# Autodesk Inventor assembly: Robot4
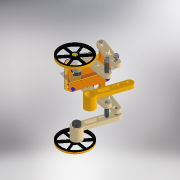
[picture p0: Inventor's stored thumbnail of the model, 180x180]
Saved by Autodesk Inventor 2021 (Build 250183000, 183)
## iProperties
Created: 2024-04-10
Part Number: Robot4
Document SubType Name: Assembly
Designer: Martin
Author: Martin
## Documents named in this file (17)
- C:\Users\ASUS\OneDrive - Universidad de Antioquia\2024-1\Robótica\Proyecto\CAD\op1\Robot4.iam
- C:\Users\ASUS\OneDrive - Universidad de Antioquia\2024-1\Robótica\Proyecto\CAD\op1\BaseEnsamble.iam
- C:\Users\ASUS\OneDrive - Universidad de Antioquia\2024-1\Robótica\Proyecto\CAD\op1\EslabonCodoTrasero.ipt
- C:\Users\ASUS\OneDrive - Universidad de Antioquia\2024-1\Robótica\Proyecto\CAD\op1\EslabonRodillaCadera.ipt
- C:\Users\ASUS\OneDrive - Universidad de Antioquia\2024-1\Robótica\Proyecto\CAD\op1\Llana.ipt
- C:\Users\ASUS\OneDrive - Universidad de Antioquia\2024-1\Robótica\Proyecto\CAD\37d-gearmotor-19-30-encoder.ipt
- C:\Users\ASUS\OneDrive - Universidad de Antioquia\2024-1\Robótica\Proyecto\CAD\Resorte.ipt
- C:\Users\ASUS\Documents\Inventor\Content Center Files\R2021\en-US\GB_T 276-94 60000-RS and LS\Bearing 61900-LS GB_T 276-94.ipt
- C:\Users\ASUS\Documents\Inventor\Content Center Files\R2021\en-US\AS 1111\AS 1111 - M8 x 90.ipt
- C:\Users\ASUS\Documents\Inventor\Content Center Files\R2021\en-US\ISO 1207(2)\ISO 1207 - M8 x 50.ipt
- C:\Users\ASUS\Documents\Inventor\Content Center Files\R2021\en-US\AS 1112 (2)\AS 1112 - M8  Type 5.ipt
- C:\Users\ASUS\OneDrive - Universidad de Antioquia\2024-1\Robótica\Proyecto\CAD\op1\EslabonCodoTrasero_MIR2.ipt
- C:\Users\ASUS\OneDrive - Universidad de Antioquia\2024-1\Robótica\Proyecto\CAD\op1\EslabonRodillaCadera_MIR2.ipt
- C:\Users\ASUS\OneDrive - Universidad de Antioquia\2024-1\Robótica\Proyecto\CAD\op1\EslabonRuedaRodilla_MIR2.ipt
- C:\Users\ASUS\OneDrive - Universidad de Antioquia\2024-1\Robótica\Proyecto\CAD\op1\Llana_MIR1.ipt
- C:\Users\ASUS\OneDrive - Universidad de Antioquia\2024-1\Robótica\Proyecto\CAD\37d-gearmotor-19-30-encoder_MIR2.ipt
- C:\Users\ASUS\OneDrive - Universidad de Antioquia\2024-1\Robótica\Proyecto\CAD\Resorte_MIR3.ipt
## Components (39 placed, 16 different names)
1. BaseEnsamble:1 [sub-assembly] — Mate:11, Mate:12, Mate:13, Insert:1
2. EslabonCodoTrasero:1 — Mate:13, Mate:22, Mate:23, Mate:28, Mate:29, Insert:2, Insert:3
3. EslabonRodillaCadera:1 — Mate:11, Mate:12, Mate:14, Mate:15
4. Llana:1 — Mate:5
5. 37d-gearmotor-19-30-encoder:1 — Mate:5
6. Resorte:1
7. Rolling bearing GB/T 276-1994 Type 60000-RS and LS 61900-LS:1 — Mate:14, Mate:15
8. Rolling bearing GB/T 276-1994 Type 60000-RS and LS 61900-LS:2
9. Rolling bearing GB/T 276-1994 Type 60000-RS and LS 61900-LS:3 — Mate:22, Mate:23, Mate:31
10. Rolling bearing GB/T 276-1994 Type 60000-RS and LS 61900-LS:4
11. Rolling bearing GB/T 276-1994 Type 60000-RS and LS 61900-LS:5
12. AS 1111 - Metric M8 x 90:1 — Mate:32
13. ISO 1207 M8 x 50:1 — Mate:30
14. AS 1111 - Metric M8 x 90:2 — Mate:28, Mate:29
15. AS 1112 (2) - Metric M8  Type 5:1 — Insert:1
16. AS 1112 (2) - Metric M8  Type 5:2 — Mate:30, Mate:31
17. AS 1112 (2) - Metric M8  Type 5:3 — Insert:2
18. AS 1112 (2) - Metric M8  Type 5:4 — Insert:3
19. AS 1112 (2) - Metric M8  Type 5:5 — Mate:32
20. EslabonCodoTrasero_MIR2:1 — Mate:33, Mate:34, Mate:46, Mate:47, Mate:56, Mate:57, Insert:4, Insert:5
21. EslabonRodillaCadera_MIR2:1 — Mate:35, Mate:36, Mate:42, Mate:43
22. EslabonRuedaRodilla_MIR2:1 — Mate:33, Mate:34, Mate:35, Mate:36, Mate:37, Mate:39, Mate:40, Mate:41, Mate:44, Mate:45, Mate:48, Mate:49, Mate:50, Mate:51, Mate:52, Mate:53, Mate:54, Mate:55
23. Llana_MIR1:1 — Mate:37, Mate:38
24. 37d-gearmotor-19-30-encoder_MIR2:1 — Mate:38, Mate:39, Mate:40
25. Resorte_MIR3:1 — Mate:41
26. Rolling bearing GB/T 276-1994 Type 60000-RS and LS 61900-LS:6 — Mate:42, Mate:43
27. Rolling bearing GB/T 276-1994 Type 60000-RS and LS 61900-LS:7 — Mate:44, Mate:45
28. Rolling bearing GB/T 276-1994 Type 60000-RS and LS 61900-LS:8 — Mate:46, Mate:47, Mate:58
29. Rolling bearing GB/T 276-1994 Type 60000-RS and LS 61900-LS:9 — Mate:48, Mate:49
30. Rolling bearing GB/T 276-1994 Type 60000-RS and LS 61900-LS:10 — Mate:50, Mate:51
31. AS 1111 - Metric M8 x 90:3 — Mate:52, Mate:53, Mate:60
32. ISO 1207 M8 x 50:2 — Mate:54, Mate:55, Mate:59
33. AS 1111 - Metric M8 x 90:4 — Mate:56, Mate:57
34. AS 1112 (2) - Metric M8  Type 5:6
35. AS 1112 (2) - Metric M8  Type 5:7 — Mate:58, Mate:59
36. AS 1112 (2) - Metric M8  Type 5:8 — Insert:4
37. AS 1112 (2) - Metric M8  Type 5:9 — Insert:5
38. AS 1112 (2) - Metric M8  Type 5:10 — Mate:60
39. EslabonRuedaRodilla_MIR2:2
## Relationships (46: Mate 41, Insert 5)
- Mate:5: Llana:1 ↔ 37d-gearmotor-19-30-encoder:1
- Mate:11: BaseEnsamble:1 ↔ EslabonRodillaCadera:1
- Mate:12 (1 mm): BaseEnsamble:1 ↔ EslabonRodillaCadera:1
- Mate:13: BaseEnsamble:1 ↔ EslabonCodoTrasero:1
- Mate:14: EslabonRodillaCadera:1 ↔ Rolling bearing GB/T 276-1994 Type 60000-RS and LS 61900-LS:1
- Mate:15: EslabonRodillaCadera:1 ↔ Rolling bearing GB/T 276-1994 Type 60000-RS and LS 61900-LS:1
- Mate:22: EslabonCodoTrasero:1 ↔ Rolling bearing GB/T 276-1994 Type 60000-RS and LS 61900-LS:3
- Mate:23: EslabonCodoTrasero:1 ↔ Rolling bearing GB/T 276-1994 Type 60000-RS and LS 61900-LS:3
- Mate:28: EslabonCodoTrasero:1 ↔ AS 1111 - Metric M8 x 90:2
- Mate:29: EslabonCodoTrasero:1 ↔ AS 1111 - Metric M8 x 90:2
- Insert:1: BaseEnsamble:1 ↔ AS 1112 (2) - Metric M8  Type 5:1
- Mate:30: ISO 1207 M8 x 50:1 ↔ AS 1112 (2) - Metric M8  Type 5:2
- Mate:31: Rolling bearing GB/T 276-1994 Type 60000-RS and LS 61900-LS:3 ↔ AS 1112 (2) - Metric M8  Type 5:2
- Insert:2: EslabonCodoTrasero:1 ↔ AS 1112 (2) - Metric M8  Type 5:3
- Insert:3: EslabonCodoTrasero:1 ↔ AS 1112 (2) - Metric M8  Type 5:4
- Mate:32: AS 1111 - Metric M8 x 90:1 ↔ AS 1112 (2) - Metric M8  Type 5:5
- Mate:33 (10 mm): EslabonCodoTrasero_MIR2:1 ↔ EslabonRuedaRodilla_MIR2:1
- Mate:34: EslabonCodoTrasero_MIR2:1 ↔ EslabonRuedaRodilla_MIR2:1
- Mate:35 (46 mm): EslabonRodillaCadera_MIR2:1 ↔ EslabonRuedaRodilla_MIR2:1
- Mate:36: EslabonRodillaCadera_MIR2:1 ↔ EslabonRuedaRodilla_MIR2:1
- Mate:37 (2 mm): EslabonRuedaRodilla_MIR2:1 ↔ Llana_MIR1:1
- Mate:38: Llana_MIR1:1 ↔ 37d-gearmotor-19-30-encoder_MIR2:1
- Mate:39: EslabonRuedaRodilla_MIR2:1 ↔ 37d-gearmotor-19-30-encoder_MIR2:1
- Mate:40: EslabonRuedaRodilla_MIR2:1 ↔ 37d-gearmotor-19-30-encoder_MIR2:1
- Mate:41: EslabonRuedaRodilla_MIR2:1 ↔ Resorte_MIR3:1
- Mate:42: EslabonRodillaCadera_MIR2:1 ↔ Rolling bearing GB/T 276-1994 Type 60000-RS and LS 61900-LS:6
- Mate:43: EslabonRodillaCadera_MIR2:1 ↔ Rolling bearing GB/T 276-1994 Type 60000-RS and LS 61900-LS:6
- Mate:44: EslabonRuedaRodilla_MIR2:1 ↔ Rolling bearing GB/T 276-1994 Type 60000-RS and LS 61900-LS:7
- Mate:45: EslabonRuedaRodilla_MIR2:1 ↔ Rolling bearing GB/T 276-1994 Type 60000-RS and LS 61900-LS:7
- Mate:46: EslabonCodoTrasero_MIR2:1 ↔ Rolling bearing GB/T 276-1994 Type 60000-RS and LS 61900-LS:8
- Mate:47: EslabonCodoTrasero_MIR2:1 ↔ Rolling bearing GB/T 276-1994 Type 60000-RS and LS 61900-LS:8
- Mate:48: EslabonRuedaRodilla_MIR2:1 ↔ Rolling bearing GB/T 276-1994 Type 60000-RS and LS 61900-LS:9
- Mate:49: EslabonRuedaRodilla_MIR2:1 ↔ Rolling bearing GB/T 276-1994 Type 60000-RS and LS 61900-LS:9
- Mate:50: EslabonRuedaRodilla_MIR2:1 ↔ Rolling bearing GB/T 276-1994 Type 60000-RS and LS 61900-LS:10
- Mate:51: EslabonRuedaRodilla_MIR2:1 ↔ Rolling bearing GB/T 276-1994 Type 60000-RS and LS 61900-LS:10
- Mate:52: EslabonRuedaRodilla_MIR2:1 ↔ AS 1111 - Metric M8 x 90:3
- Mate:53: EslabonRuedaRodilla_MIR2:1 ↔ AS 1111 - Metric M8 x 90:3
- Mate:54: EslabonRuedaRodilla_MIR2:1 ↔ ISO 1207 M8 x 50:2
- Mate:55: EslabonRuedaRodilla_MIR2:1 ↔ ISO 1207 M8 x 50:2
- Mate:56: EslabonCodoTrasero_MIR2:1 ↔ AS 1111 - Metric M8 x 90:4
- Mate:57: EslabonCodoTrasero_MIR2:1 ↔ AS 1111 - Metric M8 x 90:4
- Mate:58: Rolling bearing GB/T 276-1994 Type 60000-RS and LS 61900-LS:8 ↔ AS 1112 (2) - Metric M8  Type 5:7
- Mate:59: ISO 1207 M8 x 50:2 ↔ AS 1112 (2) - Metric M8  Type 5:7
- Insert:4: EslabonCodoTrasero_MIR2:1 ↔ AS 1112 (2) - Metric M8  Type 5:8
- Insert:5: EslabonCodoTrasero_MIR2:1 ↔ AS 1112 (2) - Metric M8  Type 5:9
- Mate:60: AS 1111 - Metric M8 x 90:3 ↔ AS 1112 (2) - Metric M8  Type 5:10
